# Autodesk Inventor assembly: Assembly of Conveyor Belt
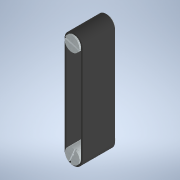
[picture p0: Inventor's stored thumbnail of the model, 180x180]
Saved by Autodesk Inventor 2022.2 (Build 262287000, 287)
## iProperties
Created: 2022-02-21
Part Number: Assembly of Conveyor Belt
Document SubType Name: Assembly
Designer: PRASHANTH
Author: PRASHANTH
## Documents named in this file (3)
- E:\BME\Autodesk Sample\Engg Exploration\Subsystem1-Conveyor Belt\Assembly of Conveyor Belt.iam
- E:\BME\Autodesk Sample\Engg Exploration\Subsystem1-Conveyor Belt\Conveyor Belt New.ipt
- E:\BME\Autodesk Sample\Engg Exploration\Subsystem1-Conveyor Belt\Conveyor Belt Shaft.ipt
## Components (3 placed, 2 different names)
1. Conveyor Belt New:1 — Mate:1, Flush:1, Rotation/Translation:1, Mate:2, Flush:2
2. Conveyor Belt Shaft:1 — Mate:1, Flush:1, Rotation/Translation:1, Rotation:1
3. Conveyor Belt Shaft:2 — Rotation:1, Mate:2, Flush:2
## Relationships (6: Mate 2, Flush 2, RelateRotateTranslate 1, RelateRotation 1)
- Mate:1: Conveyor Belt New:1 ↔ Conveyor Belt Shaft:1
- Flush:1 (-4 mm): Conveyor Belt New:1 ↔ Conveyor Belt Shaft:1
- Rotation/Translation:1 [RelateRotateTranslate] (1 mm): Conveyor Belt New:1 ↔ Conveyor Belt Shaft:1
- Rotation:1 [RelateRotation] (1 ul): Conveyor Belt Shaft:1 ↔ Conveyor Belt Shaft:2
- Mate:2: Conveyor Belt New:1 ↔ Conveyor Belt Shaft:2
- Flush:2 (-5 mm): Conveyor Belt New:1 ↔ Conveyor Belt Shaft:2
